# Autodesk Inventor assembly: Brushless Assembly
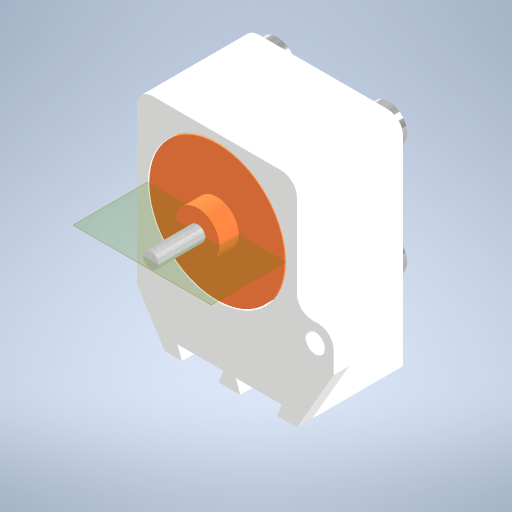
[picture p0: Inventor's stored thumbnail of the model, 512x512]
Saved by Autodesk Inventor 2024 (Build 280153000, 153)
## iProperties
Created: 2023-11-02
Part Number: Brushless Assembly
Document SubType Name: Assembly
Designer: CJ110
Author: CJ110
## Documents named in this file (4)
- D:\GitHub\Vault-1\CAD\WCRL\V1\Brushless Assembly.iam
- D:\GitHub\Vault-1\CAD\WCRL\V1\Brushless 2622 2600KV.ipt
- D:\GitHub\Vault-1\CAD\WCRL\V1\Brushless Motor Mount.ipt
- D:\GitHub\Vault-1\CAD\WCRL\V1\Brushless Motor Seat.ipt
## Components (3 placed, 3 different names)
1. Brushless 2622 2600KV:1 — Mate:1, Mate:2, Flush:1
2. Brushless Motor Mount:1 — Mate:1, Mate:2
3. Brushless Motor Seat:1 — Flush:1
## Relationships (3: Mate 2, Flush 1)
- Mate:1: Brushless 2622 2600KV:1 ↔ Brushless Motor Mount:1
- Mate:2: Brushless 2622 2600KV:1 ↔ Brushless Motor Mount:1
- Flush:1: Brushless 2622 2600KV:1 ↔ Brushless Motor Seat:1
